# Autodesk Inventor assembly: New_hinge_assembly_presentation
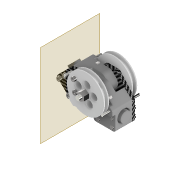
[picture p0: Inventor's stored thumbnail of the model, 180x180]
Saved by Autodesk Inventor 2022 (Build 260153000, 153)
## iProperties
Created: 2022-07-14
Part Number: New_hinge_assembly_presentation
Document SubType Name: Assembly
Designer: dell
Mass: 13.3107 g
Surface Area: 105.527 cm^2
Volume: 13.3107 cm^3
Density: 1 g/cm^3
Author: dell
## Documents named in this file (7)
- D:\xxxx\Uni\Part IV\MECHENG_700\Part_IV_project_CAD\Bird_skeleton_prototypes\Wing_drone_V1\Bird_wing_V2\New_hinge_assembly_presentation.iam
- D:\xxxx\Uni\Part IV\MECHENG_700\Part_IV_project_CAD\Bird_skeleton_prototypes\Wing_drone_V1\Bird_wing_V2\New_hinge.ipt
- D:\xxxx\Uni\Part IV\MECHENG_700\Part_IV_project_CAD\Bird_skeleton_prototypes\Wing_drone_V1\Bird_wing_V2\New_hinge_plate.ipt
- D:\xxxx\Uni\Part IV\MECHENG_700\Part_IV_project_CAD\Bird_skeleton_prototypes\Wing_drone_V1\Bird_wing_V2\New_coupling_pulley_p1.ipt
- D:\xxxx\Uni\Part IV\MECHENG_700\Part_IV_project_CAD\Bird_skeleton_prototypes\Wing_drone_V1\Bird_wing_V2\New_hinge_assembly.iam
- D:\xxxx\Uni\Part IV\MECHENG_700\Part_IV_project_CAD\Bird_skeleton_prototypes\Wing_drone_V1\Bird_wing_V2\M4_hinge_bolt.ipt
- D:\xxxx\Uni\Part IV\MECHENG_700\Part_IV_project_CAD\Bird_skeleton_prototypes\Wing_drone_V1\Bird_wing_V2\M4_nut.ipt
## Components (7 placed, 6 different names)
1. New_hinge:2 — Mate:3, Mate:4, Mate:5
2. New_hinge_plate:3 — Mate:3, Mate:4, Mate:5, Mate:12, Mate:13, Mate:14
3. New_coupling_pulley_p1:2 — Mate:12, Mate:13, Mate:14
4. New_hinge_assembly:1 [sub-assembly] — Mate:15, Mate:16, Mate:20, Angle:1
5. New_hinge_assembly:2 [sub-assembly] — Mate:15, Mate:16, Mate:17, Mate:18
6. M4_hinge_bolt:1 — Mate:17, Mate:18, Mate:19
7. M4_nut:1 — Mate:19, Mate:20
## Relationships (13: Mate 12, Angle 1)
- Mate:3: New_hinge:2 ↔ New_hinge_plate:3
- Mate:4: New_hinge:2 ↔ New_hinge_plate:3
- Mate:5: New_hinge:2 ↔ New_hinge_plate:3
- Mate:12: New_hinge_plate:3 ↔ New_coupling_pulley_p1:2
- Mate:13: New_hinge_plate:3 ↔ New_coupling_pulley_p1:2
- Mate:14: New_hinge_plate:3 ↔ New_coupling_pulley_p1:2
- Mate:15: New_hinge_assembly:1 ↔ New_hinge_assembly:2
- Mate:16: New_hinge_assembly:1 ↔ New_hinge_assembly:2
- Mate:17: New_hinge_assembly:2 ↔ M4_hinge_bolt:1
- Mate:18: New_hinge_assembly:2 ↔ M4_hinge_bolt:1
- Mate:19: M4_hinge_bolt:1 ↔ M4_nut:1
- Mate:20: New_hinge_assembly:1 ↔ M4_nut:1
- Angle:1 (225 deg): New_hinge_assembly:1
